# Autodesk Inventor assembly: Chwytak
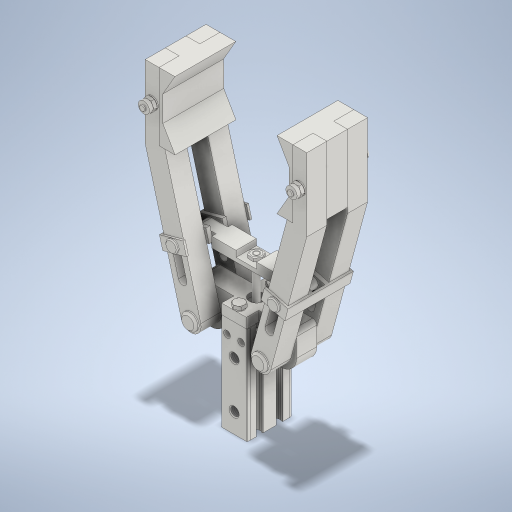
[picture p0: Inventor's stored thumbnail of the model, 512x512]
Saved by Autodesk Inventor 2024.1 (Build 281209000, 209)
## iProperties
Created: 2024-05-13
Part Number: Chwytak
Document SubType Name: Assembly
Designer: Krzysiu
Mass: 467.499 g
Surface Area: 438.26 cm^2
Volume: 68.7069 cm^3
Density: 6.80424 g/cm^3
Author: Krzysiu
## Documents named in this file (29)
- C:\Users\Krzysiu\OneDrive\Dokumenty\Inventor\Chwytak.iam
- C:\Users\Krzysiu\OneDrive\Dokumenty\Inventor\Część ramienia chwytaka.ipt
- C:\Users\Krzysiu\OneDrive\Dokumenty\Inventor\Szczęka chwytaka.ipt
- C:\Users\Krzysiu\OneDrive\Dokumenty\Inventor\Część ramienia chwytaka_MIR1.ipt
- C:\Users\Krzysiu\OneDrive\Dokumenty\Inventor\Podstawa chwytaka.ipt
- C:\Users\Krzysiu\OneDrive\Dokumenty\Inventor\Przenośnik chwytaka.ipt
- C:\Users\Krzysiu\OneDrive\Dokumenty\Inventor\Część ramienia chwytaka_MIR2.ipt
- C:\Users\Krzysiu\OneDrive\Dokumenty\Inventor\Szczęka chwytaka_MIR.ipt
- C:\Users\Krzysiu\OneDrive\Dokumenty\Inventor\Część ramienia chwytaka_MIR1_MIR.ipt
- C:\Users\Krzysiu\Documents\Inventor\Content Center Files\R2024\pl-PL\AS 1427(01)\AS 1427 - M3 x 35(3).ipt
- C:\Users\Krzysiu\Documents\Inventor\Content Center Files\R2024\pl-PL\AS 1237 (2.1)\AS 1237 - 3.ipt
- C:\Users\Krzysiu\Documents\Inventor\Content Center Files\R2024\pl-PL\AS 1285  (T1-7)\AS 1285 - M3(2).ipt
- C:\Users\Krzysiu\Documents\Inventor\4674228 DPDM-15---(h).ipt
- C:\Users\Krzysiu\Documents\Inventor\4674228 DPDM-15---(r).ipt
- C:\Users\Krzysiu\Documents\Inventor\ISO 4035 M3(F).ipt
- C:\Users\Krzysiu\OneDrive\Dokumenty\Inventor\Suwak chwytaka.ipt
- C:\Users\Krzysiu\OneDrive\Dokumenty\Inventor\Suwak chwytaka_MIR.ipt
- C:\Users\Krzysiu\Documents\Inventor\Content Center Files\R2024\pl-PL\AS 1237 (2.1)\AS 1237 - 2,5.ipt
- C:\Users\Krzysiu\Documents\Inventor\Content Center Files\R2024\pl-PL\AS 1110\AS 1110 - M2,5 x 10.ipt
- C:\Users\Krzysiu\OneDrive\Dokumenty\Inventor\Chwytak\Design Accelerator\Połączenie sworzniowe1.iam
- C:\Users\Krzysiu\OneDrive\Dokumenty\Inventor\Chwytak\Design Accelerator\Połączenie sworzniowe2.iam
- C:\Users\Krzysiu\OneDrive\Dokumenty\Inventor\Chwytak\Design Accelerator\Połączenie sworzniowe3.iam
- C:\Users\Krzysiu\OneDrive\Dokumenty\Inventor\Chwytak\Design Accelerator\Połączenie sworzniowe4.iam
- C:\Users\Krzysiu\OneDrive\Dokumenty\Inventor\Chwytak\AIP\FEA\eqcajm24g.fins
- C:\Users\Krzysiu\OneDrive\Dokumenty\Inventor\Chwytak\AIP\FEA\eqcajm24g.fsat
- C:\Users\Krzysiu\OneDrive\Dokumenty\Inventor\Chwytak\AIP\FEA\eqcajm24g.ftes
- C:\Users\Krzysiu\OneDrive\Dokumenty\Inventor\Chwytak\AIP\FEA\eqcajm24g.fwiz
- C:\Users\Krzysiu\OneDrive\Dokumenty\Inventor\Chwytak\AIP\FEA\eqcajm24h.fmsh
- C:\Users\Krzysiu\OneDrive\Dokumenty\Inventor\Chwytak\AIP\FEA\eqcajm24i.fres
## Components (28 placed, 19 different names)
1. Część ramienia chwytaka:2 — Sztywne:5, Zestawiające:4, Obrotowe:2, Zestawiające:37, Zestawiające:38
2. Szczęka chwytaka:1 — Sztywne:2, Sztywne:5
3. Część ramienia chwytaka_MIR1:1 — Sztywne:2, Zestawiające:1, Zestawiające:2, Zestawiające:3, Zestawiające:24
4. Podstawa chwytaka:1 — Obrotowe:1, Zestawiające:19, Zestawiające:22, Obrotowe:2, Sztywne:9, Zestawiające:29, Zestawiające:30, Zestawiające:31, Zestawiające:32
5. Przenośnik chwytaka:1 — Obrotowe:7, Obrotowe:8, Zestawiające:25, Zestawiające:26, Zestawiające:27, Obrotowe:10, Obrotowe:11
6. Część ramienia chwytaka_MIR2:1 — Sztywne:3, Zestawiające:8, Zestawiające:28, Zestawiające:39, Zestawiające:40
7. Szczęka chwytaka_MIR:1 — Sztywne:3, Sztywne:4
8. Część ramienia chwytaka_MIR1_MIR:1 — Sztywne:4, Zestawiające:5, Zestawiające:6, Zestawiające:7, Obrotowe:1
9. AS 1427 - Metryczny M3 x 35:1 — Zestawiające:1, Zestawiające:2
10. AS 1237 (2.1) 3:1 — Zestawiające:3, Zestawiające:4, Wstawiające:1
11. AS 1285 (T1-7) - Metryczny M3:1 — Wstawiające:1
12. AS 1427 - Metryczny M3 x 35:2 — Zestawiające:5, Zestawiające:6
13. AS 1237 (2.1) 3:2 — Zestawiające:7, Zestawiające:8, Wstawiające:2
14. AS 1285 (T1-7) - Metryczny M3:2 — Wstawiające:2
15. 4674228 DPDM-15---(h):1 — Sztywne:9
16. 4674228 DPDM-15---(r):1
17. ISO 4035 M3(F):1 — Obrotowe:8
18. ISO 4035 M3(F):2 — Obrotowe:7
19. Suwak chwytaka:1 — Zestawiające:24, Zestawiające:35, Zestawiające:36, Obrotowe:11
20. Suwak chwytaka_MIR:1 — Zestawiające:28, Obrotowe:10, Zestawiające:33, Zestawiające:34
21. AS 1237 (2.1) 2,5:1 — Zestawiające:29, Zestawiające:30, Wstawiające:3
22. AS 1110 - Metryczny M2,5 x 10:1 — Wstawiające:3
23. AS 1237 (2.1) 2,5:2 — Zestawiające:31, Zestawiające:32, Wstawiające:4
24. AS 1110 - Metryczny M2,5 x 10:2 — Wstawiające:4
25. Połączenie sworzniowe:1 [sub-assembly] — Zestawiające:33, Zestawiające:34
26. Połączenie sworzniowe:2 [sub-assembly] — Zestawiające:35, Zestawiające:36
27. Połączenie sworzniowe:3 [sub-assembly] — Zestawiające:37, Zestawiające:38
28. Połączenie sworzniowe:4 [sub-assembly] — Zestawiające:39, Zestawiające:40
## Relationships (53: Mate 35, RevoluteJoint 6, WeldJoint 5, Insert 4, Angle 2, Flush 1)
- Sztywne:2 [WeldJoint]: Szczęka chwytaka:1 ↔ Część ramienia chwytaka_MIR1:1
- Sztywne:3 [WeldJoint]: Część ramienia chwytaka_MIR2:1 ↔ Szczęka chwytaka_MIR:1
- Sztywne:4 [WeldJoint]: Szczęka chwytaka_MIR:1 ↔ Część ramienia chwytaka_MIR1_MIR:1
- Sztywne:5 [WeldJoint]: Część ramienia chwytaka:2 ↔ Szczęka chwytaka:1
- Zestawiające:1 [Mate]: Część ramienia chwytaka_MIR1:1 ↔ AS 1427 - Metryczny M3 x 35:1
- Zestawiające:2 [Mate]: Część ramienia chwytaka_MIR1:1 ↔ AS 1427 - Metryczny M3 x 35:1
- Zestawiające:3 [Mate]: Część ramienia chwytaka_MIR1:1 ↔ AS 1237 (2.1) 3:1
- Zestawiające:4 [Mate]: Część ramienia chwytaka:2 ↔ AS 1237 (2.1) 3:1
- Wstawiające:1 [Insert]: AS 1237 (2.1) 3:1 ↔ AS 1285 (T1-7) - Metryczny M3:1
- Zestawiające:5 [Mate]: Część ramienia chwytaka_MIR1_MIR:1 ↔ AS 1427 - Metryczny M3 x 35:2
- Zestawiające:6 [Mate]: Część ramienia chwytaka_MIR1_MIR:1 ↔ AS 1427 - Metryczny M3 x 35:2
- Zestawiające:7 [Mate]: Część ramienia chwytaka_MIR1_MIR:1 ↔ AS 1237 (2.1) 3:2
- Zestawiające:8 [Mate]: Część ramienia chwytaka_MIR2:1 ↔ AS 1237 (2.1) 3:2
- Wstawiające:2 [Insert]: AS 1237 (2.1) 3:2 ↔ AS 1285 (T1-7) - Metryczny M3:2
- [Mate]: 4674228 DPDM-15---(h):1 ↔ 4674228 DPDM-15---(r):1
- [Mate]: 4674228 DPDM-15---(h):1 ↔ 4674228 DPDM-15---(r):1
- [Angle] (0 deg): 4674228 DPDM-15---(h):1 ↔ 4674228 DPDM-15---(r):1
- [Mate]: 4674228 DPDM-15---(r):1 ↔ ISO 4035 M3(F):1
- [Flush]: 4674228 DPDM-15---(r):1 ↔ ISO 4035 M3(F):2
- [Mate]: 4674228 DPDM-15---(r):1 ↔ ISO 4035 M3(F):2
- [Angle] (0 deg): 4674228 DPDM-15---(r):1 ↔ ISO 4035 M3(F):2
- Obrotowe:7 [RevoluteJoint]: Przenośnik chwytaka:1 ↔ ISO 4035 M3(F):2
- Obrotowe:8 [RevoluteJoint]: Przenośnik chwytaka:1 ↔ ISO 4035 M3(F):1
- Obrotowe:1 [RevoluteJoint] (-0.1 mm): Podstawa chwytaka:1 ↔ Część ramienia chwytaka_MIR1_MIR:1
- Zestawiające:17 [Mate]
- Zestawiające:18 [Mate]
- Zestawiające:19 [Mate]: Podstawa chwytaka:1
- Zestawiające:20 [Mate]
- Zestawiające:21 [Mate]
- Zestawiające:22 [Mate]: Podstawa chwytaka:1
- Obrotowe:2 [RevoluteJoint] (0.1 mm): Część ramienia chwytaka:2 ↔ Podstawa chwytaka:1
- Zestawiające:24 [Mate] (0.1 mm): Część ramienia chwytaka_MIR1:1 ↔ Suwak chwytaka:1
- Zestawiające:25 [Mate]: Przenośnik chwytaka:1
- Zestawiające:26 [Mate]: Przenośnik chwytaka:1
- Zestawiające:27 [Mate]: Przenośnik chwytaka:1
- Zestawiające:28 [Mate] (0.1 mm): Część ramienia chwytaka_MIR2:1 ↔ Suwak chwytaka_MIR:1
- Obrotowe:10 [RevoluteJoint] (0.1 mm): Przenośnik chwytaka:1 ↔ Suwak chwytaka_MIR:1
- Sztywne:9 [WeldJoint]: Podstawa chwytaka:1 ↔ 4674228 DPDM-15---(h):1
- Zestawiające:29 [Mate]: Podstawa chwytaka:1 ↔ AS 1237 (2.1) 2,5:1
- Zestawiające:30 [Mate]: Podstawa chwytaka:1 ↔ AS 1237 (2.1) 2,5:1
- Wstawiające:3 [Insert]: AS 1237 (2.1) 2,5:1 ↔ AS 1110 - Metryczny M2,5 x 10:1
- Zestawiające:31 [Mate]: Podstawa chwytaka:1 ↔ AS 1237 (2.1) 2,5:2
- Zestawiające:32 [Mate]: Podstawa chwytaka:1 ↔ AS 1237 (2.1) 2,5:2
- Wstawiające:4 [Insert]: AS 1237 (2.1) 2,5:2 ↔ AS 1110 - Metryczny M2,5 x 10:2
- Zestawiające:33 [Mate]: Suwak chwytaka_MIR:1 ↔ Połączenie sworzniowe:1
- Zestawiające:34 [Mate]: Suwak chwytaka_MIR:1 ↔ Połączenie sworzniowe:1
- Zestawiające:35 [Mate]: Suwak chwytaka:1 ↔ Połączenie sworzniowe:2
- Zestawiające:36 [Mate]: Suwak chwytaka:1 ↔ Połączenie sworzniowe:2
- Zestawiające:37 [Mate]: Część ramienia chwytaka:2 ↔ Połączenie sworzniowe:3
- Zestawiające:38 [Mate]: Część ramienia chwytaka:2 ↔ Połączenie sworzniowe:3
- Zestawiające:39 [Mate]: Część ramienia chwytaka_MIR2:1 ↔ Połączenie sworzniowe:4
- Zestawiające:40 [Mate]: Część ramienia chwytaka_MIR2:1 ↔ Połączenie sworzniowe:4
- Obrotowe:11 [RevoluteJoint] (0.1 mm): Przenośnik chwytaka:1 ↔ Suwak chwytaka:1
## Named parameters: sa_0 = 1959, sa_1 = 1959, sa_2 = 1959, sa_3 = 1959, Finish1_Area = 247.49, Finish2_Area = 247.49, Finish3_Area = 411.484, Finish4_Area = 437.519
note: some values were not read from the file. Shown as the stored number, unit unknown: "sa_0", "sa_1", "sa_2", "sa_3", "Finish1_Area", "Finish2_Area", "Finish3_Area", "Finish4_Area".
